# Autodesk Inventor assembly: Wobbler Assembly
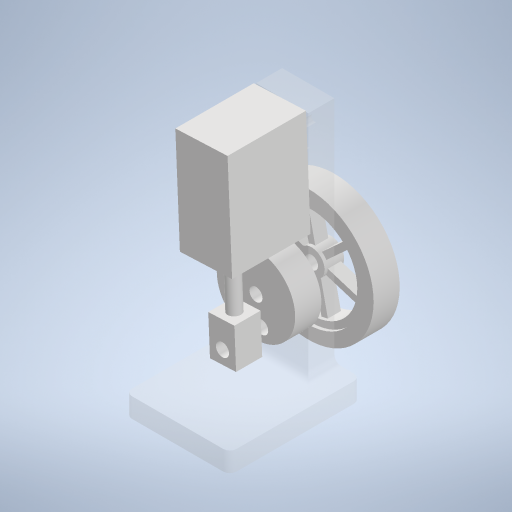
[picture p0: Inventor's stored thumbnail of the model, 512x512]
Saved by Autodesk Inventor 2023 (Build 270158000, 158)
## iProperties
Created: 2022-12-28
Part Number: Wobbler Assembly
Document SubType Name: Assembly
Designer: tgr41
Author: tgr41
## Documents named in this file (6)
- C:\Users\tgr41\OneDrive\Documents\Repositories\Steam-Engine\Cast Wobbler\Wobbler Assembly.iam
- C:\Users\tgr41\OneDrive\Documents\Repositories\Steam-Engine\Cast Wobbler\Crank.ipt
- C:\Users\tgr41\OneDrive\Documents\Repositories\Steam-Engine\Cast Wobbler\Cylinder.ipt
- C:\Users\tgr41\OneDrive\Documents\Repositories\Steam-Engine\Cast Wobbler\Flywheel.ipt
- C:\Users\tgr41\OneDrive\Documents\Repositories\Steam-Engine\Cast Wobbler\Piston Assembly.ipt
- C:\Users\tgr41\OneDrive\Documents\Repositories\Steam-Engine\Cast Wobbler\Based.ipt
## Components (5 placed, 5 different names)
1. Crank:1 — Mate:4, Mate:7, Angle:1, Mate:10
2. Cylinder:1 — Mate:6, Mate:8, Angle:2, Mate:11, Mate:12
3. Flywheel:1 — Mate:4, Mate:5, Mate:9, Angle:1
4. Based:1 — Mate:5, Mate:6, Mate:7, Mate:8, Mate:9, Angle:2
5. Piston Assembly:1 — Mate:10, Mate:11, Mate:12
## Relationships (11: Mate 9, Angle 2)
- Mate:4: Crank:1 ↔ Flywheel:1
- Mate:5: Flywheel:1 ↔ Based:1
- Mate:6: Cylinder:1 ↔ Based:1
- Mate:7: Crank:1 ↔ Based:1
- Mate:8: Cylinder:1 ↔ Based:1
- Mate:9: Flywheel:1 ↔ Based:1
- Angle:1 (0 deg): Crank:1 ↔ Flywheel:1
- Angle:2 (0 deg): Cylinder:1 ↔ Based:1
- Mate:10: Crank:1 ↔ Piston Assembly:1
- Mate:11: Cylinder:1 ↔ Piston Assembly:1
- Mate:12: Cylinder:1 ↔ Piston Assembly:1
